# Autodesk Inventor assembly: 00_Linear_Stage_NEMA11_100mm_china
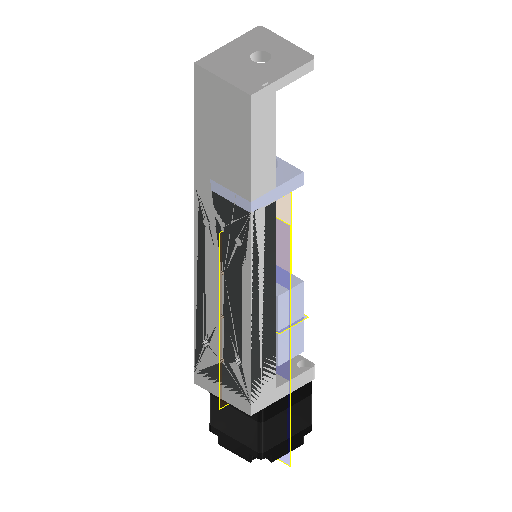
[picture p0: Inventor's stored thumbnail of the model, 512x512]
Saved by Autodesk Inventor 2022 (Build 260153000, 153)
## iProperties
Created: 2021-07-29
Part Number: 00_Linear_Stage_NEMA11_100mm_china
Document SubType Name: Assembly
Designer: diederichbenedict
Vendor: Taobao
Mass: 114.038 g
Surface Area: 468.34 cm^2
Volume: 86.3759 cm^3
Density: 1.32025 g/cm^3
Catalog Web Link: https://item.taobao.com/item.htm?spm=a1z09.2.0.0.7b072e8dkrjIPP&id=677495843151&_u=h1hhfjuv59a8
Description: Ask Haoran for Help
Sending System: SolidWorks 2021
Last Author: Albert
Last Saved: 2021-07-29
Author: diederichbenedict
## Documents named in this file (9)
- C:\Users\diederichbenedict\Dropbox\Dokumente\Promotion\PROJECTS\openUC2-CAD\INVENTOR\00_Linear_Stage_NEMA11_100mm_china.iam
- C:\Users\diederichbenedict\Dropbox\Dokumente\Promotion\PROJECTS\openUC2-CAD\INVENTOR\Base.ipt
- C:\Users\diederichbenedict\Dropbox\Dokumente\Promotion\PROJECTS\openUC2-CAD\INVENTOR\Wall_Back.ipt
- C:\Users\diederichbenedict\Dropbox\Dokumente\Promotion\PROJECTS\openUC2-CAD\INVENTOR\Wall_Front.ipt
- C:\Users\diederichbenedict\Dropbox\Dokumente\Promotion\PROJECTS\openUC2-CAD\INVENTOR\Actuator_MGN9.ipt
- C:\Users\diederichbenedict\Dropbox\Dokumente\Promotion\PROJECTS\openUC2-CAD\INVENTOR\Actuator_MGN9C.ipt
- C:\Users\diederichbenedict\Dropbox\Dokumente\Promotion\PROJECTS\openUC2-CAD\INVENTOR\Carriage.ipt
- C:\Users\diederichbenedict\Dropbox\Dokumente\Promotion\PROJECTS\openUC2-CAD\INVENTOR\Nema11.ipt
- C:\Users\diederichbenedict\Dropbox\Dokumente\Promotion\PROJECTS\openUC2-CAD\INVENTOR\Actuator_movable_100mm.ipt
## Components (8 placed, 8 different names)
1. Base:1
2. Wall_Back:1
3. Wall_Front:1
4. Actuator_MGN9:1 — Passend:1, Passend:2, Fluchtend:2
5. Actuator_MGN9C:1 — Fluchtend:1, Passend:1, Passend:3, Passend:4
6. Carriage:1 — Passend:3, Passend:4, Winkel:1
7. Nema11:1
8. Actuator_movable — Fluchtend:1, Passend:2, Winkel:1, Fluchtend:2
## Relationships (7: Mate 4, Flush 2, Angle 1)
- Fluchtend:1 [Flush]: Actuator_MGN9C:1 ↔ Actuator_movable
- Passend:1 [Mate]: Actuator_MGN9:1 ↔ Actuator_MGN9C:1
- Passend:2 [Mate]: Actuator_MGN9:1 ↔ Actuator_movable
- Passend:3 [Mate]: Actuator_MGN9C:1 ↔ Carriage:1
- Passend:4 [Mate]: Actuator_MGN9C:1 ↔ Carriage:1
- Winkel:1 [Angle] (0 deg): Carriage:1 ↔ Actuator_movable
- Fluchtend:2 [Flush]: Actuator_MGN9:1 ↔ Actuator_movable
